# Autodesk Inventor assembly: Linear actuator
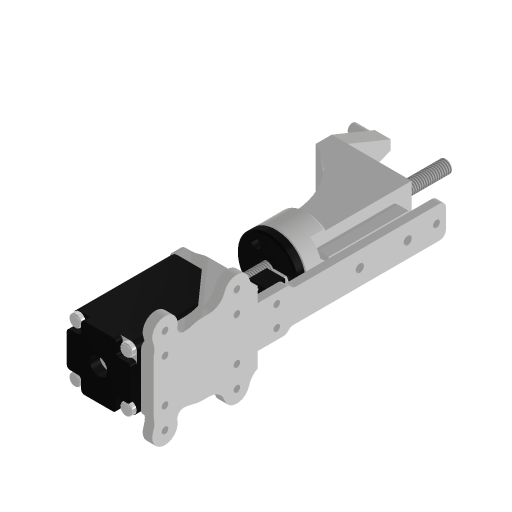
[picture p0: Inventor's stored thumbnail of the model, 512x512]
Saved by Autodesk Inventor 2023 (Build 270158000, 158)
## iProperties
Created: 2022-03-01
Part Number: Linear actuator
Document SubType Name: Assembly
Designer: ferrerx
Author: ferrerx
## Documents named in this file (8)
- C:\Users\ferrerx\Documents\GitHub\Cell_stretcher_8DOF\Design files\Mechanics\Linear actuator.iam
- C:\Users\ferrerx\Documents\GitHub\Cell_stretcher_8DOF\Design files\Mechanics\Motor holder.ipt
- C:\Users\ferrerx\Documents\GitHub\Cell_stretcher_8DOF\Design files\Mechanics\Nema 8.ipt
- C:\Users\ferrerx\Documents\GitHub\Cell_stretcher_8DOF\Design files\Mechanics\Limit switch.ipt
- C:\Users\ferrerx\Documents\GitHub\Cell_stretcher_8DOF\Design files\Mechanics\BSP10-25 bottom.iam
- C:\Users\ferrerx\Documents\GitHub\Cell_stretcher_8DOF\Design files\Mechanics\BSP10-25 top.iam
- C:\Users\ferrerx\Documents\GitHub\Cell_stretcher_8DOF\Design files\Mechanics\Nut.ipt
- C:\Users\ferrerx\Documents\GitHub\Cell_stretcher_8DOF\Design files\Mechanics\Cart.ipt
## Components (7 placed, 7 different names)
1. Motor holder:1 — Mate:1, Mate:2, Mate:3, Mate:14, Mate:17, Mate:18, Mate:19, Angle:1, Mate:22, Mate:23
2. Nema 8:1 — Mate:1, Mate:2, Mate:3, Mate:21
3. Limit switch:1 — Mate:14, Mate:22, Mate:23, Flush:1
4. BSP10-25 bottom:1 [sub-assembly] — Mate:17, Mate:18, Mate:19, Mate:20
5. BSP10-25 top:1 [sub-assembly] — Mate:20, Angle:1, Mate:27
6. Nut:1 — Mate:21, Mate:24, Mate:25, Mate:26
7. Cart:1 — Mate:24, Mate:25, Mate:26, Mate:27
## Relationships (17: Mate 15, Angle 1, Flush 1)
- Mate:1: Motor holder:1 ↔ Nema 8:1
- Mate:2: Motor holder:1 ↔ Nema 8:1
- Mate:3: Motor holder:1 ↔ Nema 8:1
- Mate:14: Motor holder:1 ↔ Limit switch:1
- Mate:17: Motor holder:1 ↔ BSP10-25 bottom:1
- Mate:18: Motor holder:1 ↔ BSP10-25 bottom:1
- Mate:19: Motor holder:1 ↔ BSP10-25 bottom:1
- Mate:20: BSP10-25 bottom:1 ↔ BSP10-25 top:1
- Angle:1 (0 deg): Motor holder:1 ↔ BSP10-25 top:1
- Mate:21: Nema 8:1 ↔ Nut:1
- Mate:22: Motor holder:1 ↔ Limit switch:1
- Mate:23: Motor holder:1 ↔ Limit switch:1
- Mate:24: Nut:1 ↔ Cart:1
- Mate:25 (0.266 mm): Nut:1 ↔ Cart:1
- Mate:26: Nut:1 ↔ Cart:1
- Mate:27: BSP10-25 top:1 ↔ Cart:1
- Flush:1 (1.7 mm): Limit switch:1
